# Autodesk Inventor assembly: клешня сбока
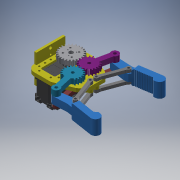
[picture p0: Inventor's stored thumbnail of the model, 180x180]
Saved by Autodesk Inventor 2019 (Build 230136000, 136)
## iProperties
Created: 2019-08-18
Part Number: клешня сбока
Material: Типовые
Document SubType Name: Assembly
Designer: Петров Иван
Author: Петров Иван
## Documents named in this file (9)
- E:\IVAN\Kvantoriada2019\optimal_gripper\hardware\КВ33.044.200 - Сборка зажима.iam
- E:\IVAN\Kvantoriada2019\optimal_gripper\hardware\КВ33.044.201 - Опора зажимного механизма.ipt
- E:\IVAN\Kvantoriada2019\optimal_gripper\hardware\КВ33.044.202 -Прихват.ipt
- E:\IVAN\Kvantoriada2019\optimal_gripper\hardware\КВ33.044.205 - Рычаг приводной 17 зубьев.ipt
- E:\IVAN\Kvantoriada2019\optimal_gripper\hardware\КВ33.044.206 - Рычаг приводной 16 зубьев.ipt
- E:\IVAN\Kvantoriada2019\optimal_gripper\hardware\КВ33.044.204 -Рычаг тонкий.ipt
- E:\IVAN\Kvantoriada2019\optimal_gripper\hardware\КВ33.044.203 - Рычаг толстый.ipt
- E:\IVAN\Kvantoriada2019\optimal_gripper\hardware\Стандартные изделия\Сервомотор Dynamixel AX-12A\ax-12a.iam
- E:\IVAN\Kvantoriada2019\optimal_gripper\hardware\КВ33.044.102 - Колесо зубчатое сервомотора.ipt
## Components (13 placed, 8 different names)
1. КВ33.044.201 - Опора зажимного механизма:1 — Совмещение:11, Совмещение:14, Совмещение:17, Совмещение:18, Совмещение:19, Совмещение:21, Совмещение:23, Совмещение:24, Совмещение:25, Совмещение:27, Совмещение:28, Совмещение:29, Совмещение:34, Совмещение:35, Совмещение:37, Совмещение:38
2. КВ33.044.202 -Прихват:1 — Совмещение:12, Совмещение:13, Совмещение:15, Совмещение:16, Совмещение:26, Совмещение:33, Совмещение:36
3. КВ33.044.202 -Прихват:2 — Совмещение:9, Совмещение:10, Совмещение:20, Совмещение:22, Совмещение:32, Совмещение:39
4. КВ33.044.204 -Рычаг тонкий:1 — Совмещение:9, Совмещение:10, Совмещение:11
5. КВ33.044.204 -Рычаг тонкий:2 — Совмещение:12, Совмещение:13, Совмещение:14
6. КВ33.044.204 -Рычаг тонкий:3 — Совмещение:15, Совмещение:16, Совмещение:17
7. КВ33.044.204 -Рычаг тонкий:4 — Совмещение:18, Совмещение:19, Совмещение:20
8. КВ33.044.203 - Рычаг толстый:1 — Совмещение:24, Совмещение:25, Совмещение:26, Совмещение:33
9. КВ33.044.203 - Рычаг толстый:2 — Совмещение:21, Совмещение:22, Совмещение:23, Совмещение:32
10. ax-12a:1 [sub-assembly] — Совмещение:27, Совмещение:28, Совмещение:29, Совмещение:30, Совмещение:31
11. КВ33.044.102 - Колесо зубчатое сервомотора:1 — Совмещение:30, Совмещение:31, Направление навивки:1
12. КВ33.044.205 - Рычаг приводной 17 зубьев:1 — Совмещение:34, Совмещение:35, Совмещение:36, Направление навивки:1, Направление навивки:2
13. КВ33.044.206 - Рычаг приводной 16 зубьев:1 — Совмещение:37, Совмещение:38, Совмещение:39, Направление навивки:2
## Relationships (33: Mate 31, RelateRotation 2)
- Совмещение:9 [Mate]: КВ33.044.202 -Прихват:2 ↔ КВ33.044.204 -Рычаг тонкий:1
- Совмещение:10 [Mate]: КВ33.044.202 -Прихват:2 ↔ КВ33.044.204 -Рычаг тонкий:1
- Совмещение:11 [Mate]: КВ33.044.201 - Опора зажимного механизма:1 ↔ КВ33.044.204 -Рычаг тонкий:1
- Совмещение:12 [Mate]: КВ33.044.202 -Прихват:1 ↔ КВ33.044.204 -Рычаг тонкий:2
- Совмещение:13 [Mate]: КВ33.044.202 -Прихват:1 ↔ КВ33.044.204 -Рычаг тонкий:2
- Совмещение:14 [Mate]: КВ33.044.201 - Опора зажимного механизма:1 ↔ КВ33.044.204 -Рычаг тонкий:2
- Совмещение:15 [Mate]: КВ33.044.202 -Прихват:1 ↔ КВ33.044.204 -Рычаг тонкий:3
- Совмещение:16 [Mate]: КВ33.044.202 -Прихват:1 ↔ КВ33.044.204 -Рычаг тонкий:3
- Совмещение:17 [Mate]: КВ33.044.201 - Опора зажимного механизма:1 ↔ КВ33.044.204 -Рычаг тонкий:3
- Совмещение:18 [Mate]: КВ33.044.201 - Опора зажимного механизма:1 ↔ КВ33.044.204 -Рычаг тонкий:4
- Совмещение:19 [Mate]: КВ33.044.201 - Опора зажимного механизма:1 ↔ КВ33.044.204 -Рычаг тонкий:4
- Совмещение:20 [Mate]: КВ33.044.202 -Прихват:2 ↔ КВ33.044.204 -Рычаг тонкий:4
- Совмещение:21 [Mate]: КВ33.044.201 - Опора зажимного механизма:1 ↔ КВ33.044.203 - Рычаг толстый:2
- Совмещение:22 [Mate]: КВ33.044.202 -Прихват:2 ↔ КВ33.044.203 - Рычаг толстый:2
- Совмещение:23 [Mate]: КВ33.044.201 - Опора зажимного механизма:1 ↔ КВ33.044.203 - Рычаг толстый:2
- Совмещение:24 [Mate]: КВ33.044.201 - Опора зажимного механизма:1 ↔ КВ33.044.203 - Рычаг толстый:1
- Совмещение:25 [Mate]: КВ33.044.201 - Опора зажимного механизма:1 ↔ КВ33.044.203 - Рычаг толстый:1
- Совмещение:26 [Mate]: КВ33.044.202 -Прихват:1 ↔ КВ33.044.203 - Рычаг толстый:1
- Совмещение:27 [Mate]: КВ33.044.201 - Опора зажимного механизма:1 ↔ ax-12a:1
- Совмещение:28 [Mate]: КВ33.044.201 - Опора зажимного механизма:1 ↔ ax-12a:1
- Совмещение:29 [Mate]: КВ33.044.201 - Опора зажимного механизма:1 ↔ ax-12a:1
- Совмещение:30 [Mate]: ax-12a:1 ↔ КВ33.044.102 - Колесо зубчатое сервомотора:1
- Совмещение:31 [Mate]: ax-12a:1 ↔ КВ33.044.102 - Колесо зубчатое сервомотора:1
- Совмещение:32 [Mate]: КВ33.044.202 -Прихват:2 ↔ КВ33.044.203 - Рычаг толстый:2
- Совмещение:33 [Mate]: КВ33.044.202 -Прихват:1 ↔ КВ33.044.203 - Рычаг толстый:1
- Совмещение:34 [Mate]: КВ33.044.201 - Опора зажимного механизма:1 ↔ КВ33.044.205 - Рычаг приводной 17 зубьев:1
- Совмещение:35 [Mate]: КВ33.044.201 - Опора зажимного механизма:1 ↔ КВ33.044.205 - Рычаг приводной 17 зубьев:1
- Совмещение:36 [Mate]: КВ33.044.202 -Прихват:1 ↔ КВ33.044.205 - Рычаг приводной 17 зубьев:1
- Совмещение:37 [Mate]: КВ33.044.201 - Опора зажимного механизма:1 ↔ КВ33.044.206 - Рычаг приводной 16 зубьев:1
- Совмещение:38 [Mate]: КВ33.044.201 - Опора зажимного механизма:1 ↔ КВ33.044.206 - Рычаг приводной 16 зубьев:1
- Совмещение:39 [Mate]: КВ33.044.202 -Прихват:2 ↔ КВ33.044.206 - Рычаг приводной 16 зубьев:1
- Направление навивки:1 [RelateRotation] (1.5 ul): КВ33.044.102 - Колесо зубчатое сервомотора:1 ↔ КВ33.044.205 - Рычаг приводной 17 зубьев:1
- Направление навивки:2 [RelateRotation] (1 ul): КВ33.044.205 - Рычаг приводной 17 зубьев:1 ↔ КВ33.044.206 - Рычаг приводной 16 зубьев:1
